# Autodesk Inventor assembly: PLANTER BOX
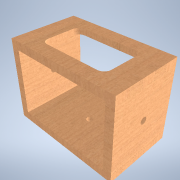
[picture p0: Inventor's stored thumbnail of the model, 180x180]
Saved by Autodesk Inventor 2021.2 (Build 252289000, 289)
## iProperties
Created: 2021-03-12
Part Number: PLANTER BOX
Document SubType Name: Assembly
Designer: 443201246
Author: 443201246
## Documents named in this file (4)
- \\SR8137CF01-FS02\StudentUsers\2025\443201246\Documents\8DT1\Planter Box\PLANTER BOX.iam
- \\SR8137CF01-FS02\StudentUsers\2025\443201246\Documents\8DT1\Planter Box\Parts\FRONT V2.ipt
- \\SR8137CF01-FS02\StudentUsers\2025\443201246\Documents\8DT1\Planter Box\Parts\SIDE V2.ipt
- \\SR8137CF01-FS02\StudentUsers\2025\443201246\Documents\8DT1\Planter Box\Parts\BACK V2.ipt
## Components (4 placed, 1 different names)
1. FRONT:1 — Flush:1, Flush:2, Flush:3, Flush:4, Flush:5, Flush:6
2. FRONT:2 — Flush:1, Flush:2, Flush:3, Flush:7, Flush:8, Flush:9
3. FRONT:3 — Flush:4, Flush:5, Flush:6
4. FRONT:4 — Flush:7, Flush:8, Flush:9
## Relationships (9: Flush 9)
- Flush:1: FRONT:1 ↔ FRONT:2
- Flush:2: FRONT:1 ↔ FRONT:2
- Flush:3: FRONT:1 ↔ FRONT:2
- Flush:4: FRONT:1 ↔ FRONT:3
- Flush:5: FRONT:1 ↔ FRONT:3
- Flush:6: FRONT:1 ↔ FRONT:3
- Flush:7: FRONT:2 ↔ FRONT:4
- Flush:8: FRONT:2 ↔ FRONT:4
- Flush:9: FRONT:2 ↔ FRONT:4
